# Autodesk Inventor assembly: short covering
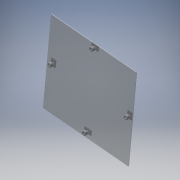
[picture p0: Inventor's stored thumbnail of the model, 180x180]
Saved by Autodesk Inventor 2016 (Build 200138000, 138)
## iProperties
Created: 2016-08-02
Part Number: short covering
Document SubType Name: Assembly
Designer: Jonathan
Author: Jonathan
## Documents named in this file (4)
- C:\Users\Jonathan\Desktop\Models\Three Panel Detector\frame\separator\short covering.iam
- C:\Users\Jonathan\Desktop\Models\Three Panel Detector\frame\separator\short covering.ipt
- C:\Users\Jonathan\Desktop\Models\Three Panel Detector\frame\brackets\m5x6.ipt
- C:\Users\Jonathan\Desktop\Models\Three Panel Detector\frame\brackets\m5TNut.ipt
## Components (9 placed, 3 different names)
1. short covering:1 — Mate:3, Mate:4, Mate:5, Angle:1, Angle:2
2. m5x6:1 — Mate:4, Mate:5, Mate:6, Angle:2
3. m5TNut:1 — Mate:3, Mate:6, Angle:1
4. m5x6:2
5. m5TNut:2
6. m5x6:3
7. m5TNut:3
8. m5x6:4
9. m5TNut:4
## Component patterns: (4 elements, first: m5x6:1 + m5TNut:1)
## Relationships (6: Mate 4, Angle 2)
- Mate:3 (2 mm): short covering:1 ↔ m5TNut:1
- Mate:4: short covering:1 ↔ m5x6:1
- Mate:5: short covering:1 ↔ m5x6:1
- Mate:6: m5x6:1 ↔ m5TNut:1
- Angle:1 (0 deg): short covering:1 ↔ m5TNut:1
- Angle:2 (0 deg): short covering:1 ↔ m5x6:1
